# Autodesk Inventor assembly: rotary control
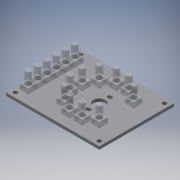
[picture p0: Inventor's stored thumbnail of the model, 180x180]
Saved by Autodesk Inventor 2016 (Build 200138000, 138)
## iProperties
Created: 2015-10-20
Part Number: rotary control
Document SubType Name: Assembly
Designer: jeremyhale
Author: jeremyhale
## Documents named in this file (3)
- \\psf\Home\Documents\Poorhouse\git\p0001\rotary control.iam
- \\psf\Home\Documents\Poorhouse\git\p0001\pcb rotary control.ipt
- \\psf\Home\Documents\Poorhouse\git\p0001\VLP-350-F.ipt
## Components (17 placed, 2 different names)
1. pcb rotary control:1 — Rotational:1, Rotational:2, Rotational:3, Rotational:4, Rotational:5, Rotational:6, Rotational:7, Rotational:8, Rotational:9, Rotational:10, Rotational:11, Rotational:12, Rotational:13, Rotational:14, Rotational:15, Rotational:16, Rotational:17, Rotational:18, Rotational:19, Rotational:20, Insert:1, Insert:2, Insert:3, Mate:1, Insert:4, Mate:2, Mate:3, Mate:4, Mate:5, Mate:6, Mate:7, Mate:8
2. VLP-350-F:1 — Rotational:1, Rotational:2
3. VLP-350-F:2 — Rotational:3, Rotational:4
4. VLP-350-F:3 — Rotational:5, Rotational:6
5. VLP-350-F:4 — Rotational:7, Rotational:8
6. VLP-350-F:5 — Rotational:13, Rotational:14
7. VLP-350-F:6 — Rotational:15, Rotational:16
8. VLP-350-F:7 — Rotational:17, Rotational:18
9. VLP-350-F:8 — Rotational:19, Rotational:20
10. VLP-350-F:9 — Rotational:11, Rotational:12
11. VLP-350-F:10 — Rotational:9, Rotational:10
12. VLP-350-F:11 — Insert:1, Insert:2
13. VLP-350-F:12 — Insert:3, Mate:1
14. VLP-350-F:13 — Insert:4, Mate:2
15. VLP-350-F:14 — Mate:3, Mate:4
16. VLP-350-F:15 — Mate:5, Mate:6
17. VLP-350-F:16 — Mate:7, Mate:8
## Relationships (32: RevoluteJoint 20, Mate 8, Insert 4)
- Rotational:1 [RevoluteJoint]: pcb rotary control:1 ↔ VLP-350-F:1
- Rotational:2 [RevoluteJoint]: pcb rotary control:1 ↔ VLP-350-F:1
- Rotational:3 [RevoluteJoint]: pcb rotary control:1 ↔ VLP-350-F:2
- Rotational:4 [RevoluteJoint]: pcb rotary control:1 ↔ VLP-350-F:2
- Rotational:5 [RevoluteJoint]: pcb rotary control:1 ↔ VLP-350-F:3
- Rotational:6 [RevoluteJoint]: pcb rotary control:1 ↔ VLP-350-F:3
- Rotational:7 [RevoluteJoint]: pcb rotary control:1 ↔ VLP-350-F:4
- Rotational:8 [RevoluteJoint]: pcb rotary control:1 ↔ VLP-350-F:4
- Rotational:9 [RevoluteJoint]: pcb rotary control:1 ↔ VLP-350-F:10
- Rotational:10 [RevoluteJoint]: pcb rotary control:1 ↔ VLP-350-F:10
- Rotational:11 [RevoluteJoint]: pcb rotary control:1 ↔ VLP-350-F:9
- Rotational:12 [RevoluteJoint]: pcb rotary control:1 ↔ VLP-350-F:9
- Rotational:13 [RevoluteJoint]: pcb rotary control:1 ↔ VLP-350-F:5
- Rotational:14 [RevoluteJoint]: pcb rotary control:1 ↔ VLP-350-F:5
- Rotational:15 [RevoluteJoint]: pcb rotary control:1 ↔ VLP-350-F:6
- Rotational:16 [RevoluteJoint]: pcb rotary control:1 ↔ VLP-350-F:6
- Rotational:17 [RevoluteJoint]: pcb rotary control:1 ↔ VLP-350-F:7
- Rotational:18 [RevoluteJoint]: pcb rotary control:1 ↔ VLP-350-F:7
- Rotational:19 [RevoluteJoint]: pcb rotary control:1 ↔ VLP-350-F:8
- Rotational:20 [RevoluteJoint]: pcb rotary control:1 ↔ VLP-350-F:8
- Insert:1: pcb rotary control:1 ↔ VLP-350-F:11
- Insert:2: pcb rotary control:1 ↔ VLP-350-F:11
- Insert:3: pcb rotary control:1 ↔ VLP-350-F:12
- Mate:1: pcb rotary control:1 ↔ VLP-350-F:12
- Insert:4: pcb rotary control:1 ↔ VLP-350-F:13
- Mate:2: pcb rotary control:1 ↔ VLP-350-F:13
- Mate:3: pcb rotary control:1 ↔ VLP-350-F:14
- Mate:4: pcb rotary control:1 ↔ VLP-350-F:14
- Mate:5: pcb rotary control:1 ↔ VLP-350-F:15
- Mate:6: pcb rotary control:1 ↔ VLP-350-F:15
- Mate:7: pcb rotary control:1 ↔ VLP-350-F:16
- Mate:8: pcb rotary control:1 ↔ VLP-350-F:16
